# Autodesk Inventor assembly: partsassembeled
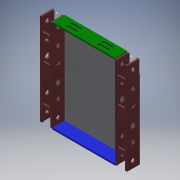
[picture p0: Inventor's stored thumbnail of the model, 180x180]
Saved by Autodesk Inventor 2017 (Build 210142000, 142)
## iProperties
Created: 2016-09-24
Part Number: partsassembeled
Document SubType Name: Assembly
Designer: vslabsal
Author: vslabsal
## Documents named in this file (5)
- C:\Users\vslabsal\Desktop\partsassembeled.iam
- C:\Users\vslabsal\Downloads\BK-BKT120-BasePlate(1).ipt
- C:\Users\vslabsal\Downloads\BT-BTK120-DriveFrameTube.ipt
- C:\Users\vslabsal\Downloads\BK-BK120-Back(2).ipt
- C:\Users\vslabsal\Downloads\BK-BKT120-Front(2).ipt
## Components (5 placed, 4 different names)
1. BK-BKT120-BasePlate(1):1 — Rigid:2, Rigid:3, Rigid:4, Rigid:5
2. BT-BTK120-DriveFrameTube:1 — Rigid:3
3. BT-BTK120-DriveFrameTube:2 — Rigid:2
4. BK-BK120-Back(2):1 — Rigid:4
5. BK-BKT120-Front(2):1 — Rigid:5
## Relationships (4: WeldJoint 4)
- Rigid:2 [WeldJoint]: BK-BKT120-BasePlate(1):1 ↔ BT-BTK120-DriveFrameTube:2
- Rigid:3 [WeldJoint]: BK-BKT120-BasePlate(1):1 ↔ BT-BTK120-DriveFrameTube:1
- Rigid:4 [WeldJoint]: BK-BKT120-BasePlate(1):1 ↔ BK-BK120-Back(2):1
- Rigid:5 [WeldJoint]: BK-BKT120-BasePlate(1):1 ↔ BK-BKT120-Front(2):1
